# Autodesk Inventor assembly: Assembly1
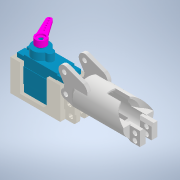
[picture p0: Inventor's stored thumbnail of the model, 180x180]
Saved by Autodesk Inventor 2020.4 (Build 244396010, 396A)
## iProperties
Created: 2021-11-02
Part Number: Assembly1
Document SubType Name: Assembly
Designer: chalo
Author: chalo
## Documents named in this file (4)
- C:\Users\chalo\OneDrive\Documents\GitHub\Interfaces-Biomedicas-2021\Gonzalo Palarea\Inventor\Ensamblaje_Final\Assembly1.iam
- C:\Users\chalo\OneDrive\Documents\GitHub\Interfaces-Biomedicas-2021\Gonzalo Palarea\Inventor\tipo2\Base_v2.ipt
- C:\Users\chalo\OneDrive\Documents\GitHub\Interfaces-Biomedicas-2021\Gonzalo Palarea\Inventor\servoconbrazo.iam
- C:\Users\chalo\OneDrive\Documents\GitHub\Interfaces-Biomedicas-2021\Gonzalo Palarea\Inventor\modificaciones prototipo 2\Metacarpo_mod2.ipt
## Components (3 placed, 3 different names)
1. Base_v2:1 — Mate:1, Insert:1, Angle:1
2. servoconbrazo:1 [sub-assembly] — Mate:1, Insert:1, Angle:1
3. Metacarpo_mod2:1
## Relationships (3: Mate 1, Insert 1, Angle 1)
- Mate:1: Base_v2:1 ↔ servoconbrazo:1
- Insert:1: Base_v2:1 ↔ servoconbrazo:1
- Angle:1 (0 deg): Base_v2:1 ↔ servoconbrazo:1
